# Autodesk Inventor assembly: miniport
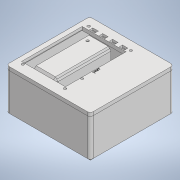
[picture p0: Inventor's stored thumbnail of the model, 180x180]
Saved by Autodesk Inventor 2020 (Build 240168000, 168)
## iProperties
Created: 2019-07-18
Part Number: miniport
Document SubType Name: Assembly
Designer: anp
Author: anp
## Documents named in this file (3)
- C:\Users\anp\Documents\Inventor\Learning\miniport.iam
- C:\Users\anp\Documents\Inventor\Learning\back.ipt
- C:\Users\anp\Documents\Inventor\Learning\cover.ipt
## Components (2 placed, 2 different names)
1. back:1 — Mate:1, Flush:2, Flush:3
2. cover:1 — Mate:1, Flush:2, Flush:3
## Relationships (3: Flush 2, Mate 1)
- Mate:1: back:1 ↔ cover:1
- Flush:2: back:1 ↔ cover:1
- Flush:3: back:1 ↔ cover:1
